# Autodesk Inventor assembly: MK4 Turret Assembly L3
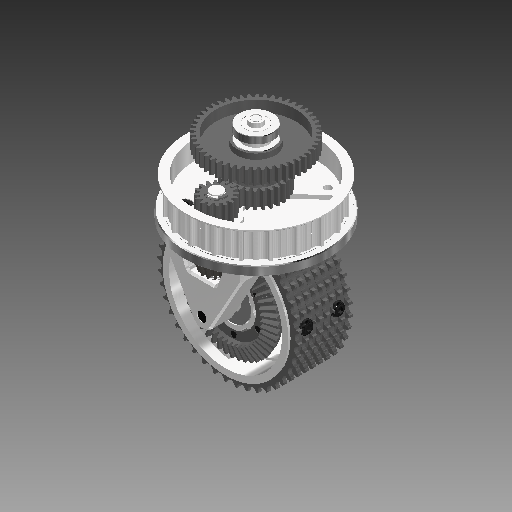
[picture p0: Inventor's stored thumbnail of the model, 512x512]
Saved by Autodesk Inventor 2025 (Build 290162010, 162A)
## iProperties
Created: 2024-07-13
Part Number: MK4 Turret Assembly L3
Document SubType Name: Assembly
Designer: rohan
Author: rohan
Revision Number: ANY
## Documents named in this file (25)
- D:\ultimate-hecker\Computer-Aided-Design\FRC-Offseason-Design-Training\Parts Library\Drivetrains\Swerve Modules\MK4\MK4 Turret Assembly L3.iam
- D:\ultimate-hecker\Computer-Aided-Design\FRC-Offseason-Design-Training\Parts Library\Drivetrains\Swerve Modules\MK4\MK4 Billet Wheel Assembly.iam
- D:\ultimate-hecker\Computer-Aided-Design\FRC-Offseason-Design-Training\Parts Library\Hardware\Fasteners\Shoulder Bolt\0.375Dia x 2.5 Shoulder Bolt.ipt
- D:\ultimate-hecker\Computer-Aided-Design\FRC-Offseason-Design-Training\Parts Library\Hardware\Fasteners\Shoulder Bolt.ipt
- D:\ultimate-hecker\Computer-Aided-Design\FRC-Offseason-Design-Training\Parts Library\Drivetrains\Swerve Modules\MK4\Wheel Mount A.ipt
- D:\ultimate-hecker\Computer-Aided-Design\FRC-Offseason-Design-Training\Parts Library\Drivetrains\Swerve Modules\MK4\Wheel Mount B.ipt
- D:\ultimate-hecker\Computer-Aided-Design\FRC-Offseason-Design-Training\Parts Library\Drivetrains\Swerve Modules\MK4\MK4 Wheel Spacer.ipt
- D:\ultimate-hecker\Computer-Aided-Design\FRC-Offseason-Design-Training\Parts Library\Power Transfer\Bearings and Bushings\Bearings\R6ZZ Bearing.ipt
- D:\ultimate-hecker\Computer-Aided-Design\FRC-Offseason-Design-Training\Parts Library\Power Transfer\Bearings and Bushings\Bearings\R8ZZ Bearing.ipt
- D:\ultimate-hecker\Computer-Aided-Design\FRC-Offseason-Design-Training\Parts Library\Power Transfer\Bearings and Bushings\Bearings\688 Bearing.ipt
- D:\ultimate-hecker\Computer-Aided-Design\FRC-Offseason-Design-Training\Parts Library\Drivetrains\Swerve Modules\MK4\MK4 Intermediate Shaft.ipt
- D:\ultimate-hecker\Computer-Aided-Design\FRC-Offseason-Design-Training\Parts Library\Hardware\Spacers\Spacers & Standoffs.ipt
- D:\ultimate-hecker\Computer-Aided-Design\FRC-Offseason-Design-Training\Parts Library\Hardware\Spacers\Spacers & Standoffs\SDS Neo Shaft Spacer 1mm.ipt
- D:\ultimate-hecker\Computer-Aided-Design\FRC-Offseason-Design-Training\Parts Library\Power Transfer\Gears (Bevel)\Bevel Gear (1545).ipt
- D:\ultimate-hecker\Computer-Aided-Design\FRC-Offseason-Design-Training\Parts Library\Drivetrains\Swerve Modules\MK3\MK3 Base Pulley.ipt
- D:\ultimate-hecker\Computer-Aided-Design\FRC-Offseason-Design-Training\Parts Library\Power Transfer\Bearings and Bushings\Bearings\6802 Bearing.ipt
- D:\ultimate-hecker\Computer-Aided-Design\FRC-Offseason-Design-Training\Parts Library\Drivetrains\Swerve Modules\MK3\MK3 Center Column.ipt
- D:\ultimate-hecker\Computer-Aided-Design\FRC-Offseason-Design-Training\Parts Library\Power Transfer\Bearings and Bushings\Bearings\A035XPO_SA035XPO Bearing.ipt
- D:\ultimate-hecker\Computer-Aided-Design\FRC-Offseason-Design-Training\Parts Library\Hardware\Fasteners\Machine Screws\1(_FS)4-20 UNCx1 Socket Head Cap Screw.ipt
- D:\ultimate-hecker\Computer-Aided-Design\FRC-Offseason-Design-Training\Parts Library\Hardware\Fasteners\Machine Screws.ipt
- D:\ultimate-hecker\Computer-Aided-Design\FRC-Offseason-Design-Training\Parts Library\Hardware\Fasteners\Machine Screws\1(_FS)4-20 UNCx0.625 Socket Head Cap Screw.ipt
- D:\ultimate-hecker\Computer-Aided-Design\FRC-Offseason-Design-Training\Parts Library\Hardware\Fasteners\E Clip.ipt
- D:\ultimate-hecker\Computer-Aided-Design\FRC-Offseason-Design-Training\Parts Library\Electronics\FRC\Sensors\CTRE Magnet for CANCoder.ipt
- D:\ultimate-hecker\Computer-Aided-Design\FRC-Offseason-Design-Training\Parts Library\Power Transfer\Gears (Hex)\50-28T 20DP Double Gear.ipt
- D:\ultimate-hecker\Computer-Aided-Design\FRC-Offseason-Design-Training\Parts Library\Power Transfer\Gears (Hex)\16T 20DP Spur Gear 375 Hex (SDS).ipt
## Components (26 placed, 21 different names)
1. MK4 Billet Wheel Assembly_50 [sub-assembly] — Rotation:2, Insert:20
2. 0.375Dia x 2.5 Shoulder Bolt:1 — Insert:1, Insert:6
3. Wheel Mount A:2 — Insert:1, Insert:2, Insert:3, Mate:14, Symmetry:1, Insert:14, Insert:15
4. Wheel Mount B:1 — Insert:6, Insert:7, Insert:9, Insert:10, Symmetry:1
5. MK4 Wheel Spacer:2 — Insert:2
6. R6ZZ Bearing:1 — Insert:3, Insert:20
7. R8ZZ Bearing:1
8. 688 Bearing:1 — Insert:7, Insert:8, Mate:19
9. MK4 Intermediate Shaft:1 — Mate:4, Mate:5, Mate:19, Mate:20, Rotation:2, Insert:18, Mate:25, Mate:26, Mate:27, Rotation:3
10. SDS Neo Shaft Spacer 1mm:1 — Insert:8, Mate:21
11. Bevel Gear (1545):1 — Mate:4, Mate:5, Mate:20, Mate:21
12. MK3 Base Pulley:1 — Insert:9, Insert:10, Mate:6, Mate:7, Mate:11, Mate:12, Mate:13, Mate:14, Mate:15, Flush:1, Mate:17, Mate:18, Insert:16, Insert:17
13. 6802 Bearing:1 — Mate:6, Mate:7
14. MK3 Center Column:2 — Mate:11, Mate:12, Mate:13, Mate:16, Insert:11, Insert:12, Mate:23, Mate:24
15. 6802 Bearing:2 — Insert:12
16. 6802 Bearing:3 — Insert:11
17. 6802 Bearing:4 — Mate:15, Mate:16, Insert:19
18. A035XPO_SA035XPO Bearing:1 — Mate:17, Mate:18
19. 1(_FS)4-20 UNCx1 Socket Head Cap Screw:1 — Insert:15
20. 1(_FS)4-20 UNCx1 Socket Head Cap Screw:2 — Insert:14
21. 1(_FS)4-20 UNCx0.625 Socket Head Cap Screw:3 — Insert:17
22. 1(_FS)4-20 UNCx0.625 Socket Head Cap Screw:4 — Insert:16
23. E Clip:1 — Insert:18
24. CTRE Magnet for CANCoder:1 — Mate:23, Mate:24
25. 50-28T 20DP Double Gear:1 — Insert:19, Rotation:3
26. 16T 20DP Spur Gear 375 Hex (SDS):1 — Mate:25, Mate:26, Mate:27
## Relationships (41: Mate 20, Insert 17, RelateRotation 2, Flush 1, Symmetry 1)
- Insert:1: 0.375Dia x 2.5 Shoulder Bolt:1 ↔ Wheel Mount A:2
- Insert:2: Wheel Mount A:2 ↔ MK4 Wheel Spacer:2
- Insert:3: Wheel Mount A:2 ↔ R6ZZ Bearing:1
- Insert:6: 0.375Dia x 2.5 Shoulder Bolt:1 ↔ Wheel Mount B:1
- Insert:7: Wheel Mount B:1 ↔ 688 Bearing:1
- Insert:8: 688 Bearing:1 ↔ SDS Neo Shaft Spacer 1mm:1
- Mate:4: MK4 Intermediate Shaft:1 ↔ Bevel Gear (1545):1
- Mate:5: MK4 Intermediate Shaft:1 ↔ Bevel Gear (1545):1
- Insert:9: Wheel Mount B:1 ↔ MK3 Base Pulley:1
- Insert:10: Wheel Mount B:1 ↔ MK3 Base Pulley:1
- Mate:6: MK3 Base Pulley:1 ↔ 6802 Bearing:1
- Mate:7: MK3 Base Pulley:1 ↔ 6802 Bearing:1
- Mate:11: MK3 Base Pulley:1 ↔ MK3 Center Column:2
- Mate:12: MK3 Base Pulley:1 ↔ MK3 Center Column:2
- Mate:13: MK3 Base Pulley:1 ↔ MK3 Center Column:2
- Mate:14: Wheel Mount A:2 ↔ MK3 Base Pulley:1
- Mate:15: MK3 Base Pulley:1 ↔ 6802 Bearing:4
- Mate:16: MK3 Center Column:2 ↔ 6802 Bearing:4
- Insert:11: MK3 Center Column:2 ↔ 6802 Bearing:3
- Insert:12: MK3 Center Column:2 ↔ 6802 Bearing:2
- Flush:1: MK3 Base Pulley:1
- Mate:17: MK3 Base Pulley:1 ↔ A035XPO_SA035XPO Bearing:1
- Mate:18: MK3 Base Pulley:1 ↔ A035XPO_SA035XPO Bearing:1
- Mate:19: 688 Bearing:1 ↔ MK4 Intermediate Shaft:1
- Mate:20: MK4 Intermediate Shaft:1 ↔ Bevel Gear (1545):1
- Mate:21: SDS Neo Shaft Spacer 1mm:1 ↔ Bevel Gear (1545):1
- Rotation:2 [RelateRotation] (0.3333 ul): MK4 Billet Wheel Assembly_50 ↔ MK4 Intermediate Shaft:1
- Symmetry:1: Wheel Mount A:2 ↔ Wheel Mount B:1
- Insert:14: Wheel Mount A:2 ↔ 1(_FS)4-20 UNCx1 Socket Head Cap Screw:2
- Insert:15: Wheel Mount A:2 ↔ 1(_FS)4-20 UNCx1 Socket Head Cap Screw:1
- Insert:16: MK3 Base Pulley:1 ↔ 1(_FS)4-20 UNCx0.625 Socket Head Cap Screw:4
- Insert:17: MK3 Base Pulley:1 ↔ 1(_FS)4-20 UNCx0.625 Socket Head Cap Screw:3
- Insert:18: MK4 Intermediate Shaft:1 ↔ E Clip:1
- Mate:23: MK3 Center Column:2 ↔ CTRE Magnet for CANCoder:1
- Mate:24: MK3 Center Column:2 ↔ CTRE Magnet for CANCoder:1
- Mate:25: MK4 Intermediate Shaft:1 ↔ 16T 20DP Spur Gear 375 Hex (SDS):1
- Mate:26: MK4 Intermediate Shaft:1 ↔ 16T 20DP Spur Gear 375 Hex (SDS):1
- Mate:27: MK4 Intermediate Shaft:1 ↔ 16T 20DP Spur Gear 375 Hex (SDS):1
- Insert:19: 6802 Bearing:4 ↔ 50-28T 20DP Double Gear:1
- Rotation:3 [RelateRotation] (0.5714 ul): MK4 Intermediate Shaft:1 ↔ 50-28T 20DP Double Gear:1
- Insert:20: MK4 Billet Wheel Assembly_50 ↔ R6ZZ Bearing:1
